# Autodesk Inventor assembly: hook_left
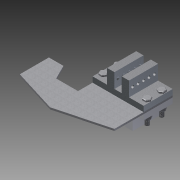
[picture p0: Inventor's stored thumbnail of the model, 180x180]
Saved by Autodesk Inventor 2011 (Build 150239000, 239)
## iProperties
Created: 2013-01-17
Part Number: hook_left
Document SubType Name: Assembly
Designer: Christopher
Author: Christopher
## Documents named in this file (6)
- F:\Users\Christopher\Documents\GitHub\2013CAD\2013 robot\forklift\frame parts\hook_left.iam
- F:\Users\Christopher\Documents\GitHub\2013CAD\2013 robot\forklift\frame parts\8020_sliders.ipt
- F:\Users\Christopher\Documents\GitHub\2013CAD\2013 robot\forklift\frame parts\plate_metal_hook.ipt
- F:\Users\Christopher\Documents\GitHub\2013CAD\2013 robot\forklift\Misc parts\nut_.25_20.ipt
- F:\Users\Christopher\Documents\GitHub\2013CAD\2013 robot\forklift\frame parts\solid_alum_chain_grabber.ipt
- F:\Users\Christopher\Documents\GitHub\2013CAD\2013 robot\forklift\Misc parts\1.5_bolt_.25_20.ipt
## Components (11 placed, 5 different names)
1. 8020_sliders:1 — Insert:7, Insert:8, Insert:9, Insert:10, Insert:17, Insert:18
2. plate_metal_hook:1 — Insert:17, Insert:18, Insert:19, Insert:20
3. nut_.25_20:1 — Insert:7
4. nut_.25_20:2 — Insert:8
5. nut_.25_20:3 — Insert:9
6. nut_.25_20:4 — Insert:10
7. solid_alum_chain_grabber:1 — Insert:13, Insert:14, Insert:15, Insert:16, Insert:19, Insert:20
8. 1.5_bolt_.25_20:1 — Insert:13
9. 1.5_bolt_.25_20:2 — Insert:14
10. 1.5_bolt_.25_20:3 — Insert:15
11. 1.5_bolt_.25_20:4 — Insert:16
## Relationships (12: Insert 12)
- Insert:7: 8020_sliders:1 ↔ nut_.25_20:1
- Insert:8: 8020_sliders:1 ↔ nut_.25_20:2
- Insert:9: 8020_sliders:1 ↔ nut_.25_20:3
- Insert:10: 8020_sliders:1 ↔ nut_.25_20:4
- Insert:13: solid_alum_chain_grabber:1 ↔ 1.5_bolt_.25_20:1
- Insert:14: solid_alum_chain_grabber:1 ↔ 1.5_bolt_.25_20:2
- Insert:15: solid_alum_chain_grabber:1 ↔ 1.5_bolt_.25_20:3
- Insert:16: solid_alum_chain_grabber:1 ↔ 1.5_bolt_.25_20:4
- Insert:17: 8020_sliders:1 ↔ plate_metal_hook:1
- Insert:18: 8020_sliders:1 ↔ plate_metal_hook:1
- Insert:19: plate_metal_hook:1 ↔ solid_alum_chain_grabber:1
- Insert:20: plate_metal_hook:1 ↔ solid_alum_chain_grabber:1
